# Autodesk Inventor assembly: Thumb Screw Assy
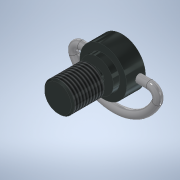
[picture p0: Inventor's stored thumbnail of the model, 180x180]
Saved by Autodesk Inventor 2020 (Build 240168000, 168)
## iProperties
Created: 2012-10-13
Part Number: Thumb Screw Assy
Document SubType Name: Assembly
Designer: Lance
Author: Lance
## Documents named in this file (3)
- C:\Users\Hesekiel\Desktop\Equatorial-Mount-MUM\Mechanika\Mechanizm elewacji Filip\CAD\manfrotto-494rc2-tripod-head.snapshot.1\Manfrotto 494RC2 - Tripod Head\Thumb Screw Assy.iam
- C:\Users\Hesekiel\Desktop\Equatorial-Mount-MUM\Mechanika\Mechanizm elewacji Filip\CAD\manfrotto-494rc2-tripod-head.snapshot.1\Manfrotto 494RC2 - Tripod Head\Thumb Screw.ipt
- C:\Users\Hesekiel\Desktop\Equatorial-Mount-MUM\Mechanika\Mechanizm elewacji Filip\CAD\manfrotto-494rc2-tripod-head.snapshot.1\Manfrotto 494RC2 - Tripod Head\Thumb Screw Handle.ipt
## Components (2 placed, 2 different names)
1. Thumb Screw:1 — Flush:1, Angle:1, Mate:1
2. Thumb Screw Handle:1 — Flush:1, Angle:1, Mate:1
## Relationships (3: Flush 1, Angle 1, Mate 1)
- Flush:1: Thumb Screw:1 ↔ Thumb Screw Handle:1
- Angle:1 (0 deg): Thumb Screw:1 ↔ Thumb Screw Handle:1
- Mate:1: Thumb Screw:1 ↔ Thumb Screw Handle:1
